# Autodesk Inventor assembly: Assembly1
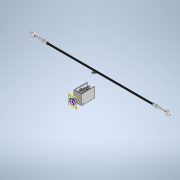
[picture p0: Inventor's stored thumbnail of the model, 180x180]
Saved by Autodesk Inventor 2022 (Build 260153000, 153)
## iProperties
Created: 2022-06-06
Part Number: Assembly1
Document SubType Name: Assembly
Designer: tecware
Author: tecware
## Documents named in this file (8)
- C:\Users\tecware\Documents\git\calibrationKit\calibrationKit_v2\wand\Assembly1.iam
- C:\Users\tecware\Documents\git\calibrationKit\calibrationKit_v2\wand\components_wand\markerWithRodEnd.ipt
- C:\Users\tecware\Documents\git\calibrationKit\calibrationKit_v2\wand\components_wand\horizontalRod.ipt
- C:\Users\tecware\Documents\git\calibrationKit\calibrationKit_v2\components\Buck Boost Converter\_xl6009_dc-dc_boost_buck.iam
- C:\Users\tecware\Documents\git\calibrationKit\calibrationKit_v2\components\SPDT Slider Switch.ipt
- C:\Users\tecware\Documents\git\calibrationKit\calibrationKit_v2\components\9V Battery\9V Battery.ipt
- C:\Users\tecware\Documents\git\calibrationKit\calibrationKit_v2\wand\Tclamp_enclosure.ipt
- C:\Users\tecware\Documents\git\calibrationKit\calibrationKit_v2\wand\tray.ipt
## Components (10 placed, 7 different names)
1. markerWithRodEnd:1 — Mate:1, Flush:1
2. markerWithRodEnd:2 — Mate:1, Flush:1, Mate:4, Mate:6
3. markerWithRodEnd:3 — Mate:3, Mate:5
4. markerWithRodEnd:4
5. horizontalRod:1 — Mate:3, Mate:4, Mate:5, Mate:6
6. _xl6009_dc-dc_boost_buck:1 [sub-assembly]
7. SPDT Slider Switch:1
8. 9V Battery:1
9. Tclamp_enclosure:1
10. tray:1
## Relationships (8: Mate 6, Flush 2)
- Mate:1: markerWithRodEnd:1 ↔ markerWithRodEnd:2
- Flush:1: markerWithRodEnd:1 ↔ markerWithRodEnd:2
- [Mate]: markerWithRodEnd:3 ↔ markerWithRodEnd:4
- [Flush]: markerWithRodEnd:3 ↔ markerWithRodEnd:4
- Mate:3: markerWithRodEnd:3 ↔ horizontalRod:1
- Mate:4: markerWithRodEnd:2 ↔ horizontalRod:1
- Mate:5: markerWithRodEnd:3 ↔ horizontalRod:1
- Mate:6: markerWithRodEnd:2 ↔ horizontalRod:1
## Named parameters: d2_d1 = 0 mm, d3_d0 = 0 mm
